# Autodesk Inventor assembly: EnsambleCapas
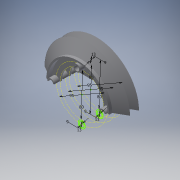
[picture p0: Inventor's stored thumbnail of the model, 180x180]
Saved by Autodesk Inventor 2019 (Build 230136000, 136)
## iProperties
Created: 2020-03-30
Part Number: EnsambleCapas
Document SubType Name: Assembly
Designer: Sergio
Author: Sergio
## Documents named in this file (3)
- C:\Users\Sergio\Documents\Innovandes\PROYECTO_GIT\EstacionMeteorologica\Diseños3D\VersionFinal\Viento\EnsambleCapas.iam
- C:\Users\Sergio\Documents\Innovandes\PROYECTO_GIT\EstacionMeteorologica\Diseños3D\VersionFinal\Viento\BaseHumedadDireccion.ipt
- C:\Users\Sergio\Documents\Innovandes\PROYECTO_GIT\EstacionMeteorologica\Diseños3D\VersionFinal\Viento\BaseHumedadDireccioncopia.ipt
## Components (3 placed, 2 different names)
1. BaseHumedadDireccion:1 — Mate:1, Mate:2, Mate:9
2. BaseHumedadDireccioncopia:1 — Mate:1, Mate:2, Mate:4, Mate:5, Mate:8, Mate:9
3. BaseHumedadDireccioncopia:2 — Mate:4, Mate:5, Mate:7, Mate:8
## Relationships (7: Mate 7)
- Mate:1: BaseHumedadDireccion:1 ↔ BaseHumedadDireccioncopia:1
- Mate:2: BaseHumedadDireccion:1 ↔ BaseHumedadDireccioncopia:1
- Mate:4: BaseHumedadDireccioncopia:1 ↔ BaseHumedadDireccioncopia:2
- Mate:5: BaseHumedadDireccioncopia:1 ↔ BaseHumedadDireccioncopia:2
- Mate:7: BaseHumedadDireccioncopia:2
- Mate:8: BaseHumedadDireccioncopia:1 ↔ BaseHumedadDireccioncopia:2
- Mate:9: BaseHumedadDireccion:1 ↔ BaseHumedadDireccioncopia:1
